# Autodesk Inventor assembly: Odompod
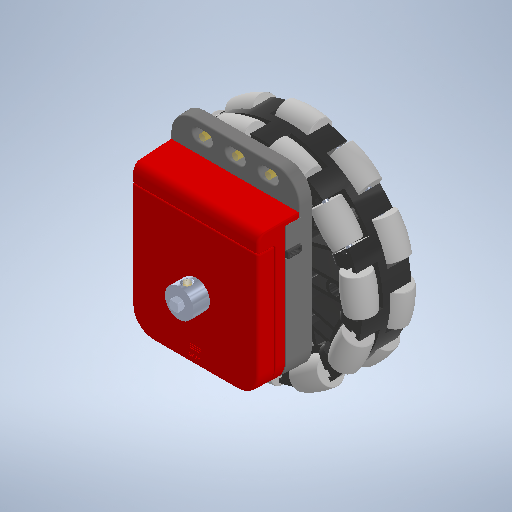
[picture p0: Inventor's stored thumbnail of the model, 512x512]
Saved by Autodesk Inventor 2025.2 (Build 292293000, 293)
## iProperties
Created: 2024-12-19
Part Number: Odompod
Document SubType Name: Assembly
Designer: joshi
Author: joshi
## Documents named in this file (10)
- C:\Users\joshi\Desktop\3388K CAD\Odompod.iam
- C:\Users\joshi\Desktop\3388K CAD\VEX Main\Electronics\Sensors\Optical Shaft Encoder.ipt
- C:\Users\joshi\Desktop\3388K CAD\VEX Main\Motion\Shaft LS\Shaft LS.ipt
- C:\Users\joshi\Desktop\3388K CAD\VEX Main\Motion\Shaft LS\Shaft LS\Shaft LS 2.5.ipt
- C:\Users\joshi\Desktop\3388K CAD\VEX Main\Motion\Shaft LS\Shaft Collar Metal\Shaft Collar No Screw.iam
- C:\Users\joshi\Desktop\3388K CAD\VEX Main\Motion\Shaft LS\Shaft Collar Metal.iam
- C:\Users\joshi\Desktop\3388K CAD\VEX Main\Motion\Spacers\Spacer Nylon .500 OD\NSpacer White .500 OD x .125.ipt
- C:\Users\joshi\Desktop\3388K CAD\VEX Main\Motion\Spacers\Spacer Nylon .500 OD.ipt
- C:\Users\joshi\Desktop\3388K CAD\VEX Main\Motion\Wheels\Omni Wheel\3.25 Omni AS, Square.iam
- C:\Users\joshi\Desktop\3388K CAD\VEX Main\Motion\Wheels\Omni Wheel.iam
## Components (6 placed, 5 different names)
1. Optical Shaft Encoder:1 — Mate:1, Mate:2, Mate:3, Mate:4
2. Shaft LS 2.5:1 — Mate:1, Mate:2, Mate:5, Mate:6
3. Shaft Collar No Screw:1 [sub-assembly] — Mate:3
4. NSpacer White .500 OD x .125:1 — Mate:4
5. 3.25 Omni AS, Square:1 [sub-assembly] — Mate:5, Mate:6, Mate:7
6. Shaft Collar No Screw:2 [sub-assembly] — Mate:7
## Relationships (7: Mate 7)
- Mate:1: Optical Shaft Encoder:1 ↔ Shaft LS 2.5:1
- Mate:2: Optical Shaft Encoder:1 ↔ Shaft LS 2.5:1
- Mate:3: Optical Shaft Encoder:1 ↔ Shaft Collar No Screw:1
- Mate:4: Optical Shaft Encoder:1 ↔ NSpacer White .500 OD x .125:1
- Mate:5: Shaft LS 2.5:1 ↔ 3.25 Omni AS, Square:1
- Mate:6: Shaft LS 2.5:1 ↔ 3.25 Omni AS, Square:1
- Mate:7: 3.25 Omni AS, Square:1 ↔ Shaft Collar No Screw:2
